# Autodesk Inventor assembly: mini Cryostat FOOT3
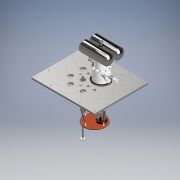
[picture p0: Inventor's stored thumbnail of the model, 180x180]
Saved by Autodesk Inventor 2018 (Build 220112000, 112)
## iProperties
Created: 2018-10-10
Part Number: mini Cryostat FOOT3
Document SubType Name: Assembly
Designer: Admin
Author: Admin
## Documents named in this file (11)
- C:\Users\Admin\Documents\Cryostat\CAD\mini Cryostat FOOT3.iam
- C:\Users\Admin\Documents\Cryostat\CAD\External Models\CH40415 24JUL14 C.ipt
- C:\Users\Admin\Documents\Cryostat\CAD\vacuum jacket long.ipt
- C:\Users\Admin\Documents\Cryostat\CAD\vacuum jacket.ipt
- C:\Users\Admin\Documents\Cryostat\CAD\Top Plate V2.2.ipt
- C:\Users\Admin\Documents\Cryostat\CAD\mini 55K stage.ipt
- C:\Users\Admin\Documents\Cryostat\CAD\foot type 3.iam
- C:\Users\Admin\Documents\Cryostat\CAD\2K8 stage mini.ipt
- C:\Users\Admin\Documents\Cryostat\CAD\Radiation Sheild 2K.ipt
- C:\Users\Admin\Documents\Cryostat\CAD\2K8 FEET.iam
- C:\Users\Admin\Documents\Cryostat\CAD\still pipe.iam
## Components (20 placed, 10 different names)
1. Top Plate V2.2:1 — Mate:16, Mate:18, Mate:19, Mate:20, Mate:21, Mate:26, Mate:57, Mate:58, Mate:59, Mate:60, Mate:61, Mate:62, Mate:89, Mate:105, Mate:106, Mate:135, Mate:136
2. CH40415 24JUL14 C:1 — Mate:16, Mate:18, Mate:26, Mate:46, Flush:1
3. vacuum jacket long:1 — Mate:7, Mate:8, Mate:9
4. vacuum jacket:1 — Mate:7, Mate:8, Mate:9, Mate:19, Mate:20, Mate:21
5. mini 55K stage:1 — Mate:46, Flush:1, Mate:49, Mate:50, Mate:52, Mate:53, Mate:54, Mate:55, Mate:56, Mate:90, Mate:91, Mate:92, Mate:93, Mate:94, Mate:97, Mate:100, Mate:102, Mate:103, Mate:104, Mate:107, Mate:108, Mate:109, Mate:110, Mate:111, Mate:112, Mate:113, Mate:114
6. foot type 3:1 [sub-assembly] — Mate:58, Mate:89, Mate:97
7. foot type 3:2 [sub-assembly] — Mate:52, Mate:57, Mate:90
8. foot type 3:3 [sub-assembly] — Mate:53, Mate:60, Mate:92
9. foot type 3:4 [sub-assembly] — Mate:54, Mate:59, Mate:91
10. foot type 3:5 [sub-assembly] — Mate:50, Mate:62, Mate:94
11. foot type 3:6 [sub-assembly] — Mate:49, Mate:61, Mate:93
12. foot type 3:7 [sub-assembly] — Mate:55, Mate:103, Mate:105
13. foot type 3:8 [sub-assembly] — Mate:56, Mate:104, Mate:106
14. 2K8 stage mini:1 — Mate:125, Mate:126, Mate:127, Mate:128, Mate:129, Mate:130, Mate:131, Mate:132
15. Radiation Sheild 2K:1 — Mate:100, Mate:102
16. 2K8 FEET:1 [sub-assembly] — Mate:107, Mate:108, Mate:127, Mate:131
17. 2K8 FEET:2 [sub-assembly] — Mate:109, Mate:113, Mate:128, Mate:132
18. 2K8 FEET:3 [sub-assembly] — Mate:110, Mate:112, Mate:125, Mate:129
19. 2K8 FEET:4 [sub-assembly] — Mate:111, Mate:114, Mate:126, Mate:130
20. still pipe:1 [sub-assembly] — Mate:135, Mate:136
## Relationships (55: Mate 54, Flush 1)
- Mate:7: vacuum jacket long:1 ↔ vacuum jacket:1
- Mate:8: vacuum jacket long:1 ↔ vacuum jacket:1
- Mate:9: vacuum jacket long:1 ↔ vacuum jacket:1
- Mate:16: Top Plate V2.2:1 ↔ CH40415 24JUL14 C:1
- Mate:18: Top Plate V2.2:1 ↔ CH40415 24JUL14 C:1
- Mate:19: Top Plate V2.2:1 ↔ vacuum jacket:1
- Mate:20: Top Plate V2.2:1 ↔ vacuum jacket:1
- Mate:21: Top Plate V2.2:1 ↔ vacuum jacket:1
- Mate:26: Top Plate V2.2:1 ↔ CH40415 24JUL14 C:1
- Mate:46: CH40415 24JUL14 C:1 ↔ mini 55K stage:1
- Flush:1: CH40415 24JUL14 C:1 ↔ mini 55K stage:1
- Mate:49: mini 55K stage:1 ↔ foot type 3:6
- Mate:50: mini 55K stage:1 ↔ foot type 3:5
- Mate:52: mini 55K stage:1 ↔ foot type 3:2
- Mate:53: mini 55K stage:1 ↔ foot type 3:3
- Mate:54: mini 55K stage:1 ↔ foot type 3:4
- Mate:55: mini 55K stage:1 ↔ foot type 3:7
- Mate:56: mini 55K stage:1 ↔ foot type 3:8
- Mate:57: Top Plate V2.2:1 ↔ foot type 3:2
- Mate:58 (2.54 mm): Top Plate V2.2:1 ↔ foot type 3:1
- Mate:59: Top Plate V2.2:1 ↔ foot type 3:4
- Mate:60: Top Plate V2.2:1 ↔ foot type 3:3
- Mate:61: Top Plate V2.2:1 ↔ foot type 3:6
- Mate:62: Top Plate V2.2:1 ↔ foot type 3:5
- Mate:89: Top Plate V2.2:1 ↔ foot type 3:1
- Mate:90: mini 55K stage:1 ↔ foot type 3:2
- Mate:91: mini 55K stage:1 ↔ foot type 3:4
- Mate:92: mini 55K stage:1 ↔ foot type 3:3
- Mate:93: mini 55K stage:1 ↔ foot type 3:6
- Mate:94: mini 55K stage:1 ↔ foot type 3:5
- Mate:97: mini 55K stage:1 ↔ foot type 3:1
- Mate:100: mini 55K stage:1 ↔ Radiation Sheild 2K:1
- Mate:102: mini 55K stage:1 ↔ Radiation Sheild 2K:1
- Mate:103: mini 55K stage:1 ↔ foot type 3:7
- Mate:104: mini 55K stage:1 ↔ foot type 3:8
- Mate:105: Top Plate V2.2:1 ↔ foot type 3:7
- Mate:106: Top Plate V2.2:1 ↔ foot type 3:8
- Mate:107: mini 55K stage:1 ↔ 2K8 FEET:1
- Mate:108: mini 55K stage:1 ↔ 2K8 FEET:1
- Mate:109: mini 55K stage:1 ↔ 2K8 FEET:2
- Mate:110: mini 55K stage:1 ↔ 2K8 FEET:3
- Mate:111: mini 55K stage:1 ↔ 2K8 FEET:4
- Mate:112: mini 55K stage:1 ↔ 2K8 FEET:3
- Mate:113: mini 55K stage:1 ↔ 2K8 FEET:2
- Mate:114: mini 55K stage:1 ↔ 2K8 FEET:4
- Mate:125: 2K8 stage mini:1 ↔ 2K8 FEET:3
- Mate:126: 2K8 stage mini:1 ↔ 2K8 FEET:4
- Mate:127: 2K8 stage mini:1 ↔ 2K8 FEET:1
- Mate:128: 2K8 stage mini:1 ↔ 2K8 FEET:2
- Mate:129: 2K8 stage mini:1 ↔ 2K8 FEET:3
- Mate:130: 2K8 stage mini:1 ↔ 2K8 FEET:4
- Mate:131: 2K8 stage mini:1 ↔ 2K8 FEET:1
- Mate:132: 2K8 stage mini:1 ↔ 2K8 FEET:2
- Mate:135: Top Plate V2.2:1 ↔ still pipe:1
- Mate:136: Top Plate V2.2:1 ↔ still pipe:1
